# Autodesk Inventor assembly: Right Side Tower Assembly
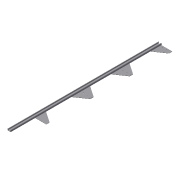
[picture p0: Inventor's stored thumbnail of the model, 180x180]
Saved by Autodesk Inventor 2015 (Build 190159000, 159)
## iProperties
Created: 2015-01-24
Part Number: Right Side Tower Assembly
Document SubType Name: Assembly
Designer: Peter
Author: Peter
## Documents named in this file (4)
- C:\Users\Tanner\Documents\GitHub\FIRST-Team-1719-CAD-Team\2015 Robot CAD\Lifter Super Structure\Tower\Side-Towers Assemblies\Right Side Tower Assembly.iam
- C:\Users\Tanner\Documents\GitHub\FIRST-Team-1719-CAD-Team\2015 Robot CAD\Lifter Super Structure\Tower\Side-Towers Assemblies\Vertical-Unistrut-Tower-75.ipt
- C:\Users\Tanner\Documents\GitHub\FIRST-Team-1719-CAD-Team\2015 Robot CAD\Lifter Super Structure\Tower\Side-Towers Assemblies\Center-Tower-Brace.ipt
- C:\Users\Tanner\Documents\GitHub\FIRST-Team-1719-CAD-Team\2015 Robot CAD\Lifter Super Structure\Tower\Side-Towers Assemblies\Corner-Tower-Brace.ipt
## Components (5 placed, 3 different names)
1. Vertical-Unistrut-Tower-75:1 — Mate:1, Flush:1, Flush:2, Mate:2, Flush:3, Mate:3, Flush:4, Mate:4, Flush:5, Flush:7, Flush:8
2. Center-Tower-Brace:1 — Mate:2, Flush:3, Mate:5
3. Corner-Tower-Brace:1 — Mate:1, Flush:1, Flush:2, Mate:5
4. Center-Tower-Brace:2 — Mate:3, Flush:4, Flush:7
5. Corner-Tower-Brace:2 — Mate:4, Flush:5, Flush:8
## Relationships (12: Flush 7, Mate 5)
- Mate:1: Vertical-Unistrut-Tower-75:1 ↔ Corner-Tower-Brace:1
- Flush:1: Vertical-Unistrut-Tower-75:1 ↔ Corner-Tower-Brace:1
- Flush:2: Vertical-Unistrut-Tower-75:1 ↔ Corner-Tower-Brace:1
- Mate:2: Vertical-Unistrut-Tower-75:1 ↔ Center-Tower-Brace:1
- Flush:3: Vertical-Unistrut-Tower-75:1 ↔ Center-Tower-Brace:1
- Mate:3: Vertical-Unistrut-Tower-75:1 ↔ Center-Tower-Brace:2
- Flush:4: Vertical-Unistrut-Tower-75:1 ↔ Center-Tower-Brace:2
- Mate:4: Vertical-Unistrut-Tower-75:1 ↔ Corner-Tower-Brace:2
- Flush:5: Vertical-Unistrut-Tower-75:1 ↔ Corner-Tower-Brace:2
- Flush:7 (-774.7 mm): Vertical-Unistrut-Tower-75:1 ↔ Center-Tower-Brace:2
- Mate:5 (269.0495 mm): Center-Tower-Brace:1 ↔ Corner-Tower-Brace:1
- Flush:8 (-311.15 mm): Vertical-Unistrut-Tower-75:1 ↔ Corner-Tower-Brace:2
## Named parameters: Lower_Center_Tower_Brace_Height = -774.7 mm
